# Autodesk Inventor assembly: jst-ph-r5
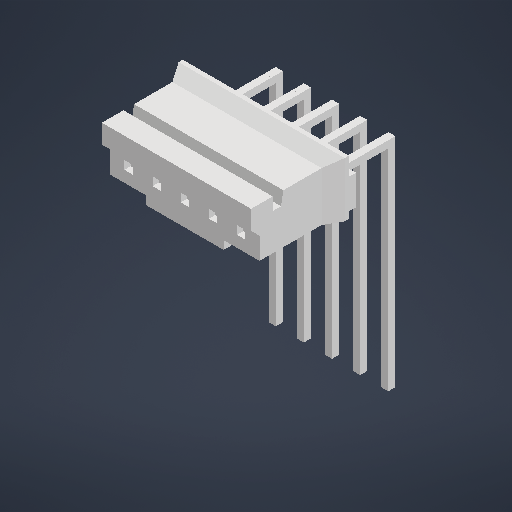
[picture p0: Inventor's stored thumbnail of the model, 512x512]
Saved by Autodesk Inventor 2025.2 (Build 292293000, 293)
## iProperties
Created: 2025-12-31
Part Number: jst-ph-r5
Document SubType Name: Assembly
Designer: sam
Author: sam
## Documents named in this file (3)
- G:\projects\primary\regulated-irrigation-system\model\asm\electronic-components\jst-ph-5p\jst-ph-r5.iam
- G:\projects\primary\regulated-irrigation-system\model\asm\electronic-components\jst-ph-5p\jst-ph-5p_wire.ipt
- G:\projects\primary\regulated-irrigation-system\model\asm\electronic-components\jst-ph-5p\jst-ph-r5.ipt
## Components (6 placed, 2 different names)
1. jst-ph-5p_wire:1 — Mate:1, Flush:1, Flush:2
2. jst-ph-r5:1 — Mate:1, Flush:1, Flush:2, Mate:2, Mate:3, Mate:4, Mate:5, Flush:3, Flush:4, Flush:5, Flush:6, Flush:7, Flush:8, Flush:9, Flush:10
3. jst-ph-5p_wire:2 — Mate:2, Flush:3, Flush:7
4. jst-ph-5p_wire:3 — Mate:3, Flush:4, Flush:8
5. jst-ph-5p_wire:4 — Mate:4, Flush:5, Flush:9
6. jst-ph-5p_wire:5 — Mate:5, Flush:6, Flush:10
## Relationships (15: Flush 10, Mate 5)
- Mate:1: jst-ph-5p_wire:1 ↔ jst-ph-r5:1
- Flush:1: jst-ph-5p_wire:1 ↔ jst-ph-r5:1
- Flush:2: jst-ph-5p_wire:1 ↔ jst-ph-r5:1
- Mate:2: jst-ph-r5:1 ↔ jst-ph-5p_wire:2
- Mate:3: jst-ph-r5:1 ↔ jst-ph-5p_wire:3
- Mate:4: jst-ph-r5:1 ↔ jst-ph-5p_wire:4
- Mate:5: jst-ph-r5:1 ↔ jst-ph-5p_wire:5
- Flush:3: jst-ph-r5:1 ↔ jst-ph-5p_wire:2
- Flush:4: jst-ph-r5:1 ↔ jst-ph-5p_wire:3
- Flush:5: jst-ph-r5:1 ↔ jst-ph-5p_wire:4
- Flush:6: jst-ph-r5:1 ↔ jst-ph-5p_wire:5
- Flush:7: jst-ph-r5:1 ↔ jst-ph-5p_wire:2
- Flush:8: jst-ph-r5:1 ↔ jst-ph-5p_wire:3
- Flush:9: jst-ph-r5:1 ↔ jst-ph-5p_wire:4
- Flush:10: jst-ph-r5:1 ↔ jst-ph-5p_wire:5
